# Autodesk Inventor assembly: Koppeltest_Halterung_Version2
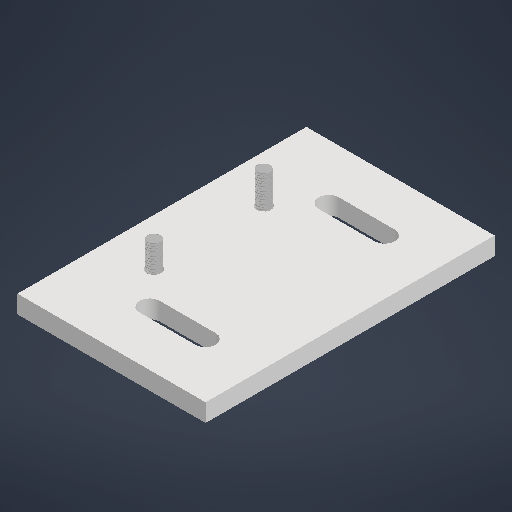
[picture p0: Inventor's stored thumbnail of the model, 512x512]
Saved by Autodesk Inventor 2027 (Build 310192060, 192F)
## iProperties
Created: 2026-06-23
Part Number: Koppeltest_Halterung_Version2
Document SubType Name: Assembly
Designer: kw
Author: kw
## Documents named in this file (3)
- C:\Users\kw\OneDrive\Documents\Uni\Masterthesis\Spezialisierungsmodul\InventorZeichnungen\Koppeltest_Halterung\Koppeltest_Halterung_massiv_RIT10.iam
- C:\Users\kw\OneDrive\Documents\Uni\Masterthesis\Spezialisierungsmodul\InventorZeichnungen\M6X20_Countersunk.ipt
- C:\Users\kw\OneDrive\Documents\Uni\Masterthesis\Spezialisierungsmodul\InventorZeichnungen\Koppeltest_Halterung\Halterung_Grundplatte_massiv.ipt
## Components (3 placed, 2 different names)
1. M6X20_Countersunk:1 — Mate:1, Flush:1
2. Halterung_Grundplatte_massiv:1 — Mate:1, Flush:1, Mate:2
3. M6X20_Countersunk:2 — Mate:2
## Relationships (3: Mate 2, Flush 1)
- Mate:1: M6X20_Countersunk:1 ↔ Halterung_Grundplatte_massiv:1
- Flush:1: M6X20_Countersunk:1 ↔ Halterung_Grundplatte_massiv:1
- Mate:2: Halterung_Grundplatte_massiv:1 ↔ M6X20_Countersunk:2
